# Autodesk Inventor assembly: Load Cell Hopper Interface
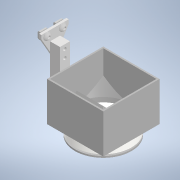
[picture p0: Inventor's stored thumbnail of the model, 180x180]
Saved by Autodesk Inventor 2022 (Build 260153000, 153)
## iProperties
Created: 2022-09-20
Part Number: Load Cell Hopper Interface
Document SubType Name: Assembly
Designer: Garrett Raker
Author: Garrett Raker
## Documents named in this file (9)
- F:\College Stuff\ATMAE Robotics\Pill Dispenser Robot\Load Cell_Hopper_Connection\Load Cell Hopper Interface.iam
- F:\College Stuff\ATMAE Robotics\Pill Dispenser Robot\Load Cell_Hopper_Connection\Load_Cell.ipt
- F:\College Stuff\ATMAE Robotics\Pill Dispenser Robot\Load Cell_Hopper_Connection\Load Cell Connector to Extrusion Bar.ipt
- F:\College Stuff\ATMAE Robotics\Pill Dispenser Robot\Load Cell_Hopper_Connection\Hopper Connector\Traingular Hopper Connector.ipt
- F:\College Stuff\ATMAE Robotics\Pill Dispenser Robot\Hoppers\M&M Hopper\M&M Hopper Assembly.iam
- F:\College Stuff\ATMAE Robotics\Pill Dispenser Robot\Load Cell_Hopper_Connection\T-Nut Block M5  Threads.ipt
- F:\College Stuff\ATMAE Robotics\Pill Dispenser Robot\Load Cell_Hopper_Connection\M4 25mm Length Flat Head Screw.ipt
- F:\College Stuff\ATMAE Robotics\Pill Dispenser Robot\Threads and Fasteners\M5 Screw 8mm length.ipt
- F:\College Stuff\ATMAE Robotics\Pill Dispenser Robot\Base Structure\2811 Series Zinc-Plated Steel Hex Nut (M4 x 0.7mm, 7mm Hex).ipt
## Components (12 placed, 8 different names)
1. Load_Cell:1 — Mate:7, Mate:8, Mate:9, Mate:10, Mate:23, Mate:24, Mate:31, Mate:32, Mate:33, Mate:34
2. Load Cell Connector to Extrusion Bar:1 — Mate:7, Mate:14, Mate:15, Mate:19, Mate:20, Mate:25, Mate:26, Mate:27, Mate:28, Mate:33, Mate:34
3. Traingular Hopper Connector:1 — Mate:8, Mate:9, Mate:10, Mate:11, Mate:12, Mate:13, Flush:1, Flush:2
4. M&M Hopper Assembly:1 [sub-assembly] — Mate:11, Mate:12, Mate:13
5. T-Nut Block M5  Threads:1 — Mate:15, Mate:20
6. T-Nut Block M5  Threads:2 — Mate:14, Mate:19
7. M4 25mm Length Flat Head Screw:1 — Mate:23, Flush:1, Mate:30
8. M4 25mm Length Flat Head Screw:2 — Mate:24, Flush:2, Mate:29
9. M5 Screw 8mm length:1 — Mate:25, Mate:27
10. M5 Screw 8mm length:2 — Mate:26, Mate:28
11. 2811 Series Zinc-Plated Steel Hex Nut (M4 x 0.7mm, 7mm Hex):1 — Mate:29, Mate:31
12. 2811 Series Zinc-Plated Steel Hex Nut (M4 x 0.7mm, 7mm Hex):2 — Mate:30, Mate:32
## Relationships (25: Mate 23, Flush 2)
- Mate:7: Load_Cell:1 ↔ Load Cell Connector to Extrusion Bar:1
- Mate:8: Load_Cell:1 ↔ Traingular Hopper Connector:1
- Mate:9: Load_Cell:1 ↔ Traingular Hopper Connector:1
- Mate:10: Load_Cell:1 ↔ Traingular Hopper Connector:1
- Mate:11: Traingular Hopper Connector:1 ↔ M&M Hopper Assembly:1
- Mate:12: Traingular Hopper Connector:1 ↔ M&M Hopper Assembly:1
- Mate:13: Traingular Hopper Connector:1 ↔ M&M Hopper Assembly:1
- Mate:14: Load Cell Connector to Extrusion Bar:1 ↔ T-Nut Block M5  Threads:2
- Mate:15: Load Cell Connector to Extrusion Bar:1 ↔ T-Nut Block M5  Threads:1
- Mate:19: Load Cell Connector to Extrusion Bar:1 ↔ T-Nut Block M5  Threads:2
- Mate:20: Load Cell Connector to Extrusion Bar:1 ↔ T-Nut Block M5  Threads:1
- Mate:23: Load_Cell:1 ↔ M4 25mm Length Flat Head Screw:1
- Mate:24: Load_Cell:1 ↔ M4 25mm Length Flat Head Screw:2
- Flush:1: Traingular Hopper Connector:1 ↔ M4 25mm Length Flat Head Screw:1
- Flush:2: Traingular Hopper Connector:1 ↔ M4 25mm Length Flat Head Screw:2
- Mate:25: Load Cell Connector to Extrusion Bar:1 ↔ M5 Screw 8mm length:1
- Mate:26: Load Cell Connector to Extrusion Bar:1 ↔ M5 Screw 8mm length:2
- Mate:27: Load Cell Connector to Extrusion Bar:1 ↔ M5 Screw 8mm length:1
- Mate:28: Load Cell Connector to Extrusion Bar:1 ↔ M5 Screw 8mm length:2
- Mate:29: M4 25mm Length Flat Head Screw:2 ↔ 2811 Series Zinc-Plated Steel Hex Nut (M4 x 0.7mm, 7mm Hex):1
- Mate:30: M4 25mm Length Flat Head Screw:1 ↔ 2811 Series Zinc-Plated Steel Hex Nut (M4 x 0.7mm, 7mm Hex):2
- Mate:31: Load_Cell:1 ↔ 2811 Series Zinc-Plated Steel Hex Nut (M4 x 0.7mm, 7mm Hex):1
- Mate:32: Load_Cell:1 ↔ 2811 Series Zinc-Plated Steel Hex Nut (M4 x 0.7mm, 7mm Hex):2
- Mate:33: Load_Cell:1 ↔ Load Cell Connector to Extrusion Bar:1
- Mate:34: Load_Cell:1 ↔ Load Cell Connector to Extrusion Bar:1
